# Autodesk Inventor assembly: assembly_arm_1
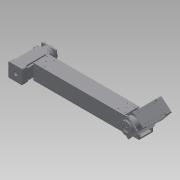
[picture p0: Inventor's stored thumbnail of the model, 180x180]
Saved by Autodesk Inventor 2017 (Build 210142000, 142)
## iProperties
Part Number: assembly_arm_1
Material: Generisch
Document SubType Name: Assembly
Designer: Max
Mass: 2675.9 g
Surface Area: 3231.18 cm^2
Volume: 1021.39 cm^3
Density: 2.61986 g/cm^3
Author: Max
## Documents named in this file (6)
- C:\Users\Max\Desktop\SENAI\robot_arm_new\assembly_arm_1.iam
- C:\Users\Max\Desktop\SENAI\robot_arm_new\dynamixel_pro_assembly.iam
- C:\Users\Max\Desktop\SENAI\robot_arm_new\cube_square_tube.ipt
- C:\Users\Max\Desktop\SENAI\robot_arm_new\square_tube.ipt
- C:\Users\Max\Desktop\SENAI\robot_arm_new\complex_frame\complex_cube.ipt
- C:\Users\Max\Desktop\SENAI\robot_arm_new\complex_frame\complex_cube_plane.ipt
## Components (6 placed, 5 different names)
1. dynamixel_pro_assembly:1 [sub-assembly] — Passend:1, Passend:2, Passend:3, Passend:4
2. cube_square_tube:1 — Passend:1, Passend:2, Passend:3, Passend:5, Passend:6, Passend:7, Passend:8
3. square_tube:1 — Passend:6, Passend:7, Passend:8, Passend:9, Passend:10, Passend:11
4. complex_cube:1 — Passend:9, Passend:10, Passend:11, Passend:14, Passend:20, Passend:21
5. complex_cube_plane:1 — Passend:14, Passend:17, Passend:18, Passend:19, Passend:20, Passend:21
6. dynamixel_pro_assembly:2 [sub-assembly] — Passend:17, Passend:18, Passend:19
## Relationships (17: Mate 17)
- Passend:1 [Mate]: dynamixel_pro_assembly:1 ↔ cube_square_tube:1
- Passend:2 [Mate]: dynamixel_pro_assembly:1 ↔ cube_square_tube:1
- Passend:3 [Mate]: dynamixel_pro_assembly:1 ↔ cube_square_tube:1
- Passend:4 [Mate]: dynamixel_pro_assembly:1
- Passend:5 [Mate]: cube_square_tube:1
- Passend:6 [Mate]: cube_square_tube:1 ↔ square_tube:1
- Passend:7 [Mate]: cube_square_tube:1 ↔ square_tube:1
- Passend:8 [Mate]: cube_square_tube:1 ↔ square_tube:1
- Passend:9 [Mate]: square_tube:1 ↔ complex_cube:1
- Passend:10 [Mate]: square_tube:1 ↔ complex_cube:1
- Passend:11 [Mate]: square_tube:1 ↔ complex_cube:1
- Passend:14 [Mate]: complex_cube:1 ↔ complex_cube_plane:1
- Passend:17 [Mate]: complex_cube_plane:1 ↔ dynamixel_pro_assembly:2
- Passend:18 [Mate]: complex_cube_plane:1 ↔ dynamixel_pro_assembly:2
- Passend:19 [Mate]: complex_cube_plane:1 ↔ dynamixel_pro_assembly:2
- Passend:20 [Mate]: complex_cube:1 ↔ complex_cube_plane:1
- Passend:21 [Mate]: complex_cube:1 ↔ complex_cube_plane:1
